# Autodesk Inventor assembly: LunaHolesSetup
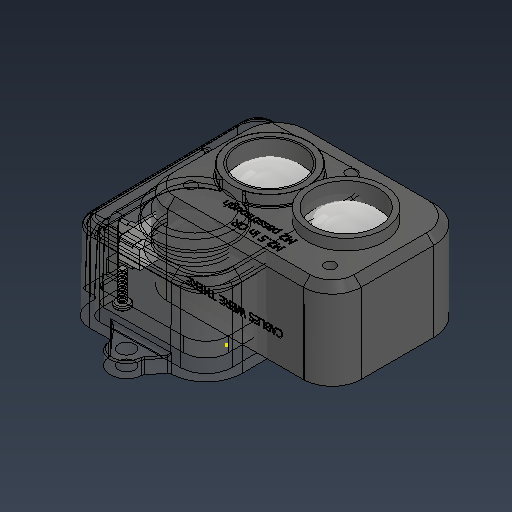
[picture p0: Inventor's stored thumbnail of the model, 512x512]
Saved by Autodesk Inventor 2026.2 (Build 302298010, 298A)
## iProperties
Created: 2026-05-03
Part Number: LunaHolesSetup
Document SubType Name: Assembly
Designer: szymo
Author: szymo
## Documents named in this file (3)
- D:\tech\robotyka\robots\evangelion-turbo\inventor-project\LunaHolesSetup.iam
- D:\tech\robotyka\robots\evangelion-turbo\inventor-project\LUNA.ipt
- D:\tech\robotyka\robots\evangelion-turbo\inventor-project\AssemBeneWake TF-LUNA\AssemBeneWake TF-LUNA\AssemBeneWake TF-LUNA.ipt
## Components (2 placed, 2 different names)
1. LUNA:1 — Flush:1, Mate:1
2. AssemBeneWake TF-LUNA:1 — Flush:1, Mate:1
## Relationships (2: Flush 1, Mate 1)
- Flush:1: LUNA:1 ↔ AssemBeneWake TF-LUNA:1
- Mate:1: LUNA:1 ↔ AssemBeneWake TF-LUNA:1
